# Autodesk Inventor assembly: DriveTrainFrameAssembly
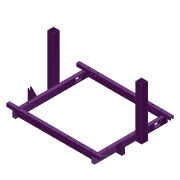
[picture p0: Inventor's stored thumbnail of the model, 180x180]
Saved by Autodesk Inventor 2012 (Build 160160000, 160)
## iProperties
Created: 2013-01-06
Part Number: DriveTrainFrameAssembly
Document SubType Name: Assembly
Designer: JesseK
Mass: 3177.66 g
Surface Area: 7638.01 cm^2
Volume: 1172.57 cm^3
Density: 2.71 g/cm^3
Author: JesseK
## Documents named in this file (5)
- Z:\UserData\Documents\Inventor\team1885frc\Robot2013\DriveTrain\DriveTrainFrameAssembly.iam
- Z:\UserData\Documents\Inventor\team1885frc\Robot2013\DriveTrain\FrameSideRail.ipt
- Z:\UserData\Documents\Inventor\team1885frc\Robot2013\DriveTrain\FrameRepresentation_FrontRear.ipt
- Z:\UserData\Documents\Inventor\team1885frc\Robot2013\DriveTrain\FrameSideBumperMounts.ipt
- Z:\UserData\Documents\Inventor\team1885frc\Robot2013\MainSupportColumn.ipt
## Components (8 placed, 4 different names)
1. FrameSideRail:1 — Flush:3, Mate:9, Flush:5, Mate:14, Mate:15, Mate:16, Mate:21, Mate:24, Flush:7, Mate:36
2. FrameSideRail:2 — Mate:13, Mate:17, Mate:18, Mate:20, Mate:26, Flush:6, Mate:34
3. FrameRepresentation_FrontRear:1 — Flush:3, Mate:9, Mate:14, Mate:18, Mate:33
4. FrameRepresentation_FrontRear:2 — Flush:5, Mate:13, Mate:15, Mate:16, Mate:17, Mate:35, Mate:37
5. FrameSideBumperMounts:2 — Mate:21, Mate:24, Mate:32
6. FrameSideBumperMounts:4 — Mate:20, Mate:26, Mate:32, Mate:33
7. MainSupportColumn:1 — Flush:7, Mate:36, Mate:37
8. MainSupportColumn:2 — Flush:6, Mate:34, Mate:35
## Relationships (21: Mate 17, Flush 4)
- Flush:3: FrameSideRail:1 ↔ FrameRepresentation_FrontRear:1
- Mate:9: FrameSideRail:1 ↔ FrameRepresentation_FrontRear:1
- Flush:5: FrameSideRail:1 ↔ FrameRepresentation_FrontRear:2
- Mate:13: FrameSideRail:2 ↔ FrameRepresentation_FrontRear:2
- Mate:14: FrameSideRail:1 ↔ FrameRepresentation_FrontRear:1
- Mate:15: FrameSideRail:1 ↔ FrameRepresentation_FrontRear:2
- Mate:16: FrameSideRail:1 ↔ FrameRepresentation_FrontRear:2
- Mate:17: FrameSideRail:2 ↔ FrameRepresentation_FrontRear:2
- Mate:18: FrameSideRail:2 ↔ FrameRepresentation_FrontRear:1
- Mate:20: FrameSideRail:2 ↔ FrameSideBumperMounts:4
- Mate:21: FrameSideRail:1 ↔ FrameSideBumperMounts:2
- Mate:24: FrameSideRail:1 ↔ FrameSideBumperMounts:2
- Mate:26: FrameSideRail:2 ↔ FrameSideBumperMounts:4
- Mate:32: FrameSideBumperMounts:2 ↔ FrameSideBumperMounts:4
- Mate:33 (152.4 mm): FrameRepresentation_FrontRear:1 ↔ FrameSideBumperMounts:4
- Flush:6: FrameSideRail:2 ↔ MainSupportColumn:2
- Mate:34: FrameSideRail:2 ↔ MainSupportColumn:2
- Mate:35 (190.5 mm): FrameRepresentation_FrontRear:2 ↔ MainSupportColumn:2
- Flush:7: FrameSideRail:1 ↔ MainSupportColumn:1
- Mate:36: FrameSideRail:1 ↔ MainSupportColumn:1
- Mate:37 (190.5 mm): FrameRepresentation_FrontRear:2 ↔ MainSupportColumn:1
